# Autodesk Inventor assembly: Assembly1
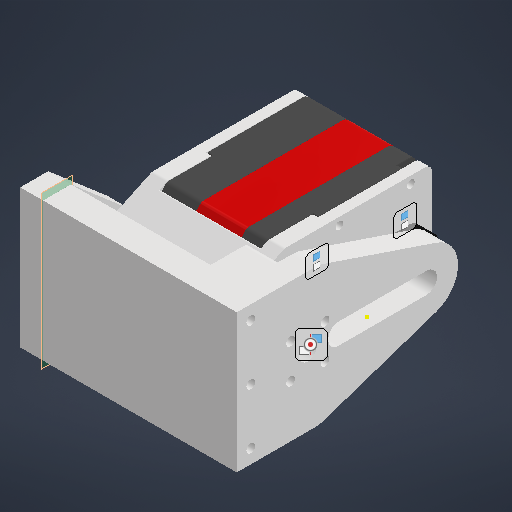
[picture p0: Inventor's stored thumbnail of the model, 512x512]
Saved by Autodesk Inventor 2026 (Build 300175000, 175)
## iProperties
Created: 2025-12-05
Part Number: Assembly1
Document SubType Name: Assembly
Designer: numai
Author: numai
## Documents named in this file (7)
- C:\Users\numai\Documents\workspace\inventor\feetech_slider_3dprint\Assembly1.iam
- C:\Users\numai\Documents\workspace\inventor\feetech_slider_3dprint\HLS3950M.ipt
- C:\Users\numai\Documents\workspace\inventor\feetech_slider_3dprint\ARRMA_1_7_25t_servo_arm.ipt
- C:\Users\numai\Documents\workspace\inventor\feetech_slider_3dprint\servo_side_plate1.ipt
- C:\Users\numai\Documents\workspace\inventor\feetech_slider_3dprint\servo_side_plate2.ipt
- C:\Users\numai\Documents\workspace\inventor\feetech_slider_3dprint\guideline.ipt
- C:\Users\numai\Documents\workspace\inventor\feetech_slider_3dprint\slider_02.ipt
## Components (6 placed, 6 different names)
1. HLS3950M:1 — メイト:1, メイト:2, フラッシュ:1, フラッシュ:2, フラッシュ:3, 角度:1
2. ARRMA_1_7_25t_servo_arm:1 — メイト:1, メイト:2, メイト:4
3. servo_side_plate1:1 — フラッシュ:1, フラッシュ:2, メイト:3
4. servo_side_plate2:1 — フラッシュ:3
5. guideline:1 — メイト:3, メイト:4, フラッシュ:4, フラッシュ:5, 角度:1
6. slider_02:1 — フラッシュ:4, フラッシュ:5
## Relationships (10: Flush 5, Mate 4, Angle 1)
- メイト:1 [Mate]: HLS3950M:1 ↔ ARRMA_1_7_25t_servo_arm:1
- メイト:2 [Mate] (0.4 mm): HLS3950M:1 ↔ ARRMA_1_7_25t_servo_arm:1
- フラッシュ:1 [Flush]: HLS3950M:1 ↔ servo_side_plate1:1
- フラッシュ:2 [Flush]: HLS3950M:1 ↔ servo_side_plate1:1
- フラッシュ:3 [Flush]: HLS3950M:1 ↔ servo_side_plate2:1
- メイト:3 [Mate]: servo_side_plate1:1 ↔ guideline:1
- メイト:4 [Mate] (1.7 mm): ARRMA_1_7_25t_servo_arm:1 ↔ guideline:1
- フラッシュ:4 [Flush]: guideline:1 ↔ slider_02:1
- フラッシュ:5 [Flush]: guideline:1 ↔ slider_02:1
- 角度:1 [Angle] (0 deg): HLS3950M:1 ↔ guideline:1
